# Autodesk Inventor assembly: Second Potential Carriage
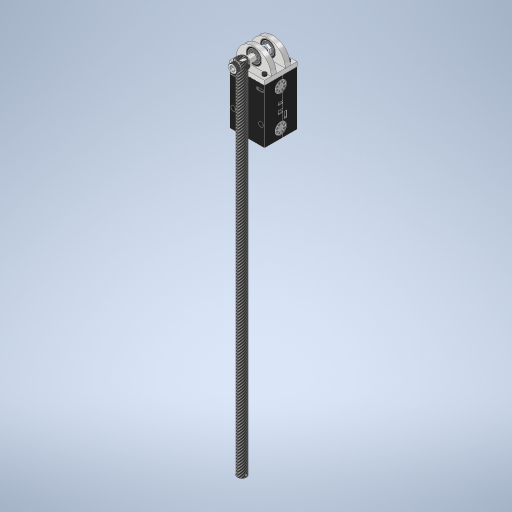
[picture p0: Inventor's stored thumbnail of the model, 512x512]
Saved by Autodesk Inventor 2023 (Build 270158000, 158)
## iProperties
Created: 2023-02-15
Part Number: Second Potential Carriage
Document SubType Name: Assembly
Designer: mbear
Author: mbear
## Documents named in this file (14)
- C:\Users\mbear\OneDrive\Documents\Inventor\Inverted Pendulum\Second Potential Carriage.iam
- C:\Users\mbear\OneDrive\Documents\Inventor\Inverted Pendulum\Carriage Design Left.ipt
- C:\Users\mbear\OneDrive\Documents\Inventor\Inverted Pendulum\Carriage Design Right.ipt
- C:\Users\mbear\OneDrive\Documents\Inventor\Inverted Pendulum\Carriage Top Second Option.ipt
- C:\Users\mbear\OneDrive\Documents\Inventor\Inverted Pendulum\Skate-Bearing.ipt
- C:\Users\mbear\OneDrive\Documents\Inventor\Inverted Pendulum\Dry Bearing.ipt
- C:\Users\mbear\OneDrive\Documents\Inventor\Inverted Pendulum\91290A169_Alloy Steel Socket Head Screw.ipt
- C:\Users\mbear\OneDrive\Documents\Inventor\Inverted Pendulum\Pendulum Tubing.ipt
- C:\Users\mbear\OneDrive\Documents\Inventor\Inverted Pendulum\Carriage Axle Design 2 Spacer.ipt
- C:\Users\mbear\OneDrive\Documents\Inventor\Inverted Pendulum\M7 Hex Nut.ipt
- C:\Users\mbear\OneDrive\Documents\Inventor\Inverted Pendulum\Hex_Socket_M3x16.ipt
- C:\Users\mbear\OneDrive\Documents\Inventor\Inverted Pendulum\M3 Nyloc Nut.ipt
- C:\Users\mbear\OneDrive\Documents\Inventor\Inverted Pendulum\M3 Square Nut.ipt
- C:\Users\mbear\OneDrive\Documents\Inventor\Inverted Pendulum\Hex_Socket_M3x14.ipt
## Components (28 placed, 13 different names)
1. Carriage Design Left:1 — Mate:1, Flush:1, Flush:2, Mate:2, Flush:3, Flush:4, Insert:18, Insert:19, Angle:7, Angle:8, Insert:20, Insert:21
2. Carriage Design Right:1 — Mate:1, Flush:1, Flush:2, Insert:3, Insert:4, Insert:5, Insert:6, Insert:16, Insert:17, Angle:5, Angle:6, Insert:22, Angle:9, Insert:23, Angle:10
3. Carriage Top Second Option:1 — Mate:2, Flush:3, Flush:4, Insert:1, Insert:2, Angle:4, Insert:12, Insert:13, Insert:14, Insert:15
4. Skate-Bearing:1 — Insert:1, Mate:3, Insert:7, Insert:8, Insert:10
5. Skate-Bearing:2 — Insert:2, Insert:9
6. Dry Bearing:1 — Insert:3
7. Dry Bearing:2 — Insert:6
8. Dry Bearing:3 — Insert:4
9. Dry Bearing:4 — Insert:5
10. Pendulum Tubing:1 — Mate:3, Flush:5, Mate:4, Flush:6, Mate:6, Angle:4
11. 91290A169_Alloy Steel Socket Head Screw:1 — Mate:4, Mate:5, Insert:7, Angle:1, Angle:2
12. Carriage Axle Design 2 Spacer:1 — Insert:8
13. M7 Hex Nut:1 — Insert:9, Angle:2, Angle:3
14. M7 Hex Nut:2 — Insert:10, Angle:3
15. Hex_Socket_M3x16:1 — Mate:6, Mate:7, Insert:11
16. M3 Nyloc Nut:1 — Insert:11
17. Hex_Socket_M3x16:2 — Insert:15
18. Hex_Socket_M3x16:3 — Insert:14
19. Hex_Socket_M3x16:4 — Insert:13
20. Hex_Socket_M3x16:5 — Insert:12
21. M3 Square Nut:1 — Insert:19, Angle:7
22. M3 Square Nut:2 — Insert:18, Angle:8
23. M3 Square Nut:3 — Insert:17, Angle:5
24. M3 Square Nut:4 — Insert:16, Angle:6
25. Hex_Socket_M3x14:1 — Insert:21
26. Hex_Socket_M3x14:2 — Insert:20
27. M3 Square Nut:5 — Insert:22, Angle:9
28. M3 Square Nut:6 — Insert:23, Angle:10
## Relationships (46: Insert 23, Angle 10, Mate 7, Flush 6)
- Mate:1: Carriage Design Left:1 ↔ Carriage Design Right:1
- Flush:1: Carriage Design Left:1 ↔ Carriage Design Right:1
- Flush:2: Carriage Design Left:1 ↔ Carriage Design Right:1
- Mate:2: Carriage Design Left:1 ↔ Carriage Top Second Option:1
- Flush:3: Carriage Design Left:1 ↔ Carriage Top Second Option:1
- Flush:4: Carriage Design Left:1 ↔ Carriage Top Second Option:1
- Insert:1: Carriage Top Second Option:1 ↔ Skate-Bearing:1
- Insert:2: Carriage Top Second Option:1 ↔ Skate-Bearing:2
- Insert:3: Carriage Design Right:1 ↔ Dry Bearing:1
- Insert:4: Carriage Design Right:1 ↔ Dry Bearing:3
- Insert:5: Carriage Design Right:1 ↔ Dry Bearing:4
- Insert:6: Carriage Design Right:1 ↔ Dry Bearing:2
- Mate:3: Skate-Bearing:1 ↔ Pendulum Tubing:1
- Flush:5 (6.35 mm): Pendulum Tubing:1
- Mate:4: Pendulum Tubing:1 ↔ 91290A169_Alloy Steel Socket Head Screw:1
- Mate:5: 91290A169_Alloy Steel Socket Head Screw:1
- Insert:7: Skate-Bearing:1 ↔ 91290A169_Alloy Steel Socket Head Screw:1
- Flush:6 (6.35 mm): Pendulum Tubing:1
- Angle:1 (0 deg): 91290A169_Alloy Steel Socket Head Screw:1
- Insert:8: Skate-Bearing:1 ↔ Carriage Axle Design 2 Spacer:1
- Insert:9: Skate-Bearing:2 ↔ M7 Hex Nut:1
- Angle:2 (0 deg): 91290A169_Alloy Steel Socket Head Screw:1 ↔ M7 Hex Nut:1
- Insert:10: Skate-Bearing:1 ↔ M7 Hex Nut:2
- Angle:3 (0 deg): M7 Hex Nut:1 ↔ M7 Hex Nut:2
- Mate:6: Pendulum Tubing:1 ↔ Hex_Socket_M3x16:1
- Mate:7: Hex_Socket_M3x16:1
- Insert:11 (-0.508 mm): Hex_Socket_M3x16:1 ↔ M3 Nyloc Nut:1
- Angle:4 (0 deg): Carriage Top Second Option:1 ↔ Pendulum Tubing:1
- Insert:12: Carriage Top Second Option:1 ↔ Hex_Socket_M3x16:5
- Insert:13: Carriage Top Second Option:1 ↔ Hex_Socket_M3x16:4
- Insert:14: Carriage Top Second Option:1 ↔ Hex_Socket_M3x16:3
- Insert:15: Carriage Top Second Option:1 ↔ Hex_Socket_M3x16:2
- Insert:16: Carriage Design Right:1 ↔ M3 Square Nut:4
- Insert:17: Carriage Design Right:1 ↔ M3 Square Nut:3
- Angle:5 (0 deg): Carriage Design Right:1 ↔ M3 Square Nut:3
- Angle:6 (0 deg): Carriage Design Right:1 ↔ M3 Square Nut:4
- Insert:18: Carriage Design Left:1 ↔ M3 Square Nut:2
- Insert:19: Carriage Design Left:1 ↔ M3 Square Nut:1
- Angle:7 (0 deg): Carriage Design Left:1 ↔ M3 Square Nut:1
- Angle:8 (0 deg): Carriage Design Left:1 ↔ M3 Square Nut:2
- Insert:20: Carriage Design Left:1 ↔ Hex_Socket_M3x14:2
- Insert:21: Carriage Design Left:1 ↔ Hex_Socket_M3x14:1
- Insert:22: Carriage Design Right:1 ↔ M3 Square Nut:5
- Angle:9 (0 deg): Carriage Design Right:1 ↔ M3 Square Nut:5
- Insert:23: Carriage Design Right:1 ↔ M3 Square Nut:6
- Angle:10 (0 deg): Carriage Design Right:1 ↔ M3 Square Nut:6
